# Autodesk Inventor assembly: 3.25 Traction AS, Circle_MIR
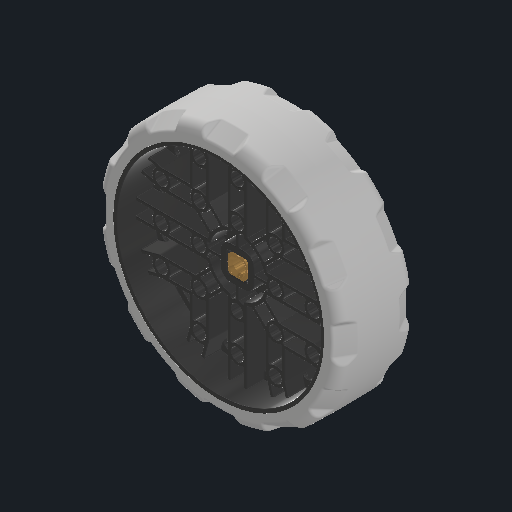
[picture p0: Inventor's stored thumbnail of the model, 512x512]
Saved by Autodesk Inventor 2024 (Build 280153000, 153)
## iProperties
Created: 2022-08-02
Part Number: 3.25 Traction AS, Circle_MIR
Document SubType Name: Assembly
Designer: macbook
Author: ylu12
## Documents named in this file (3)
- \\Mac\Home\Desktop\code\1599V-VRC\Cad\Motion\Wheels\Traction Wheel\3.25 Traction AS, Circle_MIR.iam
- \\Mac\Home\Desktop\code\1599V-VRC\Cad\Motion\Wheels\Reference Files\3.25 Traction Antistatic_MIR.ipt
- \\Mac\Home\Desktop\code\1599V-VRC\Cad\Motion\HS Shaft Adapter Circle_MIR2.ipt
## Components (2 placed, 2 different names)
1. 3.25 Traction Antistatic_MIR:1 — Mate:24, Mate:22, Mate:20
2. HS Shaft Adapter Circle_MIR2:1 — Flush:10, Mate:33, Mate:32
## Relationships (6: Flush 3, Mate 3)
- Mate:24 [Flush]: 3.25 Traction Antistatic_MIR:1
- Mate:22 [Flush]: 3.25 Traction Antistatic_MIR:1
- Mate:20: 3.25 Traction Antistatic_MIR:1
- Flush:10 (-6.35 mm): HS Shaft Adapter Circle_MIR2:1
- Mate:33: HS Shaft Adapter Circle_MIR2:1
- Mate:32: HS Shaft Adapter Circle_MIR2:1
## Named parameters: Thickness = 8.255 mm
